# Autodesk Inventor assembly: Povorot_mec.ipt
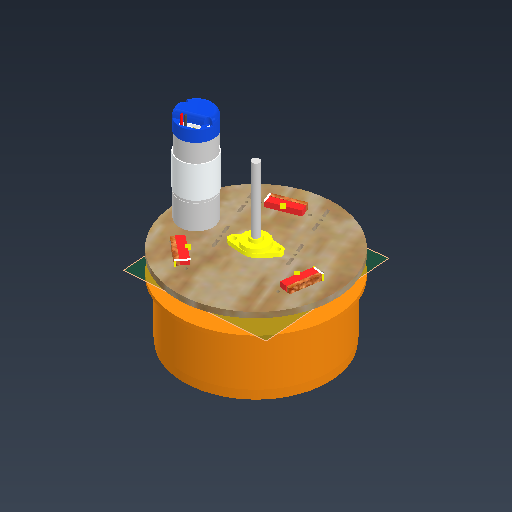
[picture p0: Inventor's stored thumbnail of the model, 512x512]
Saved by Autodesk Inventor 2023.2 (Build 272271030, 271C)
## iProperties
Created: 2023-12-24
Part Number: Povorot_mec.ipt
Document SubType Name: Assembly
Designer: Dell
Author: Dell
## Documents named in this file (15)
- D:\!project\fox_n_crow_construction\crow\rotation_block\Povorot_mec.ipt.iam
- D:\!project\fox_n_crow_construction\crow\rotation_block\Pitsco Education-739085.ipt
- D:\!project\fox_n_crow_construction\crow\rotation_block\Cap_pipes.ipt
- D:\!project\fox_n_crow_construction\crow\rotation_block\Pitsco Education-739028.ipt
- D:\!project\fox_n_crow_construction\crow\rotation_block\Fanerka.ipt
- D:\!project\fox_n_crow_construction\crow\rotation_block\Prostavka.ipt
- D:\!project\fox_n_crow_construction\crow\rotation_block\Det_podsh.ipt
- D:\!project\fox_n_crow_construction\crow\rotation_block\Podsh.ipt
- D:\!project\fox_n_crow_construction\crow\rotation_block\User Library-Bearing KFL08.ipt
- D:\!project\fox_n_crow_construction\crow\rotation_block\trubka.ipt
- D:\!project\fox_n_crow_construction\crow\rotation_block\39079_TXM-Motor Shaft Hub With Set Screw.ipt
- D:\!project\fox_n_crow_construction\crow\rotation_block\SHF8_Горизонтальный_держатель_вала.ipt
- D:\!project\fox_n_crow_construction\crow\rotation_block\ISO 14583 — M5x16-4.8.ipt
- D:\!project\fox_n_crow_construction\crow\rotation_block\ISO 7046-1 - M6 x 20_ - 4.8 - H - ISO.ipt
- D:\!project\fox_n_crow_construction\crow\rotation_block\44260_txm torquenado dc motor.ipt
## Components (22 placed, 14 different names)
1. Pitsco Education-739085:1 — Жесткий:6, Совмещение:10, Совмещение:11, Совмещение:13, Совмещение:16
2. Cap_pipes:1 — Цилиндрический:2, Совмещение:8, Совмещение:9
3. Pitsco Education-739028:1
4. Fanerka:1 — Совмещение:9, Плоский:1, Плоский:2, Плоский:3, С поворотом:3, С поворотом:4, С поворотом:5
5. Prostavka:1 — Цилиндрический:2, Совмещение:8
6. User Library-Bearing KFL08:1 — С поворотом:3, С поворотом:4
7. trubka:1 — Жесткий:6, Цилиндрический:5
8. 39079_TXM-Motor Shaft Hub With Set Screw:1
9. Винт ISO 14583:2011(E) M5x16-4.8:2
10. Винт ISO 14583:2011(E) M5x16-4.8:3
11. SHF8_Горизонтальный_держатель_вала:3 — Цилиндрический:5
12. ISO 7046-1 H M6 x 20 - 4.8 - H:1 — Совмещение:10
13. ISO 7046-1 H M6 x 20 - 4.8 - H:2 — Совмещение:11
14. ISO 7046-1 H M6 x 20 - 4.8 - H:3 — Совмещение:13
15. ISO 7046-1 H M6 x 20 - 4.8 - H:4 — Совмещение:16
16. 44260_txm torquenado dc motor:1 — С поворотом:5
17. Det_podsh:2 — С поворотом:1, Плоский:1, Плоский:2, Плоский:3
18. Podsh:1 — С поворотом:1
19. Det_podsh:3
20. Podsh:2
21. Det_podsh:4
22. Podsh:3
## Component patterns: (3 elements, first: Det_podsh:2 + Podsh:1)
## Relationships (16: Mate 6, RevoluteJoint 4, PlanarJoint 3, CylindricalJoint 2, WeldJoint 1)
- Цилиндрический:2 [CylindricalJoint]: Cap_pipes:1 ↔ Prostavka:1
- Совмещение:8 [Mate]: Cap_pipes:1 ↔ Prostavka:1
- Совмещение:9 [Mate]: Cap_pipes:1 ↔ Fanerka:1
- С поворотом:1 [RevoluteJoint]: Det_podsh:2 ↔ Podsh:1
- Плоский:1 [PlanarJoint]: Fanerka:1 ↔ Det_podsh:2
- Плоский:2 [PlanarJoint]: Fanerka:1 ↔ Det_podsh:2
- Плоский:3 [PlanarJoint]: Fanerka:1 ↔ Det_podsh:2
- Жесткий:6 [WeldJoint]: Pitsco Education-739085:1 ↔ trubka:1
- С поворотом:3 [RevoluteJoint]: Fanerka:1 ↔ User Library-Bearing KFL08:1
- С поворотом:4 [RevoluteJoint]: Fanerka:1 ↔ User Library-Bearing KFL08:1
- Цилиндрический:5 [CylindricalJoint]: trubka:1 ↔ SHF8_Горизонтальный_держатель_вала:3
- Совмещение:10 [Mate]: Pitsco Education-739085:1 ↔ ISO 7046-1 H M6 x 20 - 4.8 - H:1
- Совмещение:11 [Mate]: Pitsco Education-739085:1 ↔ ISO 7046-1 H M6 x 20 - 4.8 - H:2
- Совмещение:13 [Mate]: Pitsco Education-739085:1 ↔ ISO 7046-1 H M6 x 20 - 4.8 - H:3
- Совмещение:16 [Mate]: Pitsco Education-739085:1 ↔ ISO 7046-1 H M6 x 20 - 4.8 - H:4
- С поворотом:5 [RevoluteJoint]: Fanerka:1 ↔ 44260_txm torquenado dc motor:1
